# Autodesk Inventor assembly: 00_KES400
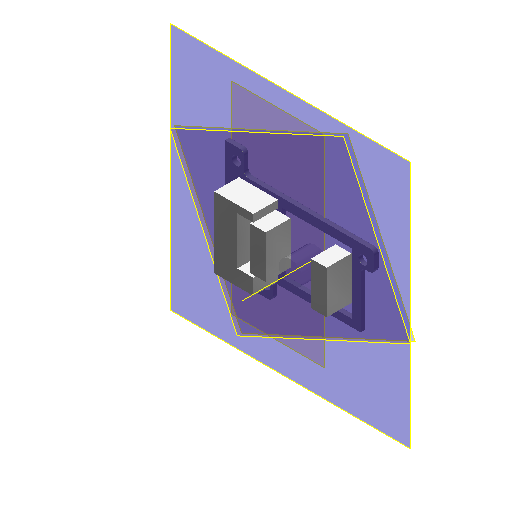
[picture p0: Inventor's stored thumbnail of the model, 512x512]
Saved by Autodesk Inventor 2022 (Build 260153000, 153)
## iProperties
Created: 2019-04-29
Part Number: 00_KES400
Document SubType Name: Assembly
Designer: diederichbenedict
Author: diederichbenedict
## Documents named in this file (4)
- C:\Users\diederichbenedict\Dropbox\Dokumente\Promotion\PROJECTS\UC2\02_CAD\INVENTOR\uc2_v3\00_KES400.iam
- C:\Users\diederichbenedict\Dropbox\Dokumente\Promotion\PROJECTS\UC2\02_CAD\INVENTOR\uc2_v3\00_KES400_Bluray_Lens.ipt
- C:\Users\diederichbenedict\Dropbox\Dokumente\Promotion\PROJECTS\UC2\02_CAD\INVENTOR\uc2_v3\00_KES_Bluray_Magnet.ipt
- C:\Users\diederichbenedict\Dropbox\Dokumente\Promotion\PROJECTS\UC2\02_CAD\INVENTOR\uc2_v3\00_KES400_Lens.ipt
## Components (3 placed, 3 different names)
1. 00_KES400_Bluray_Lens:1 — Flush:1, Flush:2, Flush:5, Flush:6
2. 00_KES_Bluray_Magnet:1 — Flush:1, Flush:2, Flush:5, Flush:7
3. 00_KES400_Lens:1 — Flush:6, Flush:7
## Relationships (5: Flush 5)
- Flush:1: 00_KES400_Bluray_Lens:1 ↔ 00_KES_Bluray_Magnet:1
- Flush:2: 00_KES400_Bluray_Lens:1 ↔ 00_KES_Bluray_Magnet:1
- Flush:5: 00_KES400_Bluray_Lens:1 ↔ 00_KES_Bluray_Magnet:1
- Flush:6: 00_KES400_Bluray_Lens:1 ↔ 00_KES400_Lens:1
- Flush:7: 00_KES_Bluray_Magnet:1 ↔ 00_KES400_Lens:1
